# Autodesk Inventor assembly: Assembly2
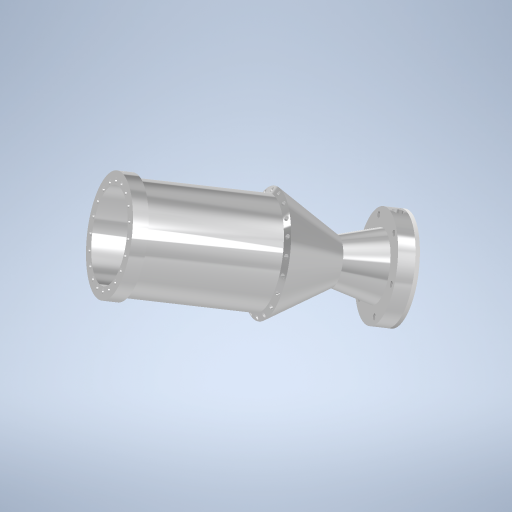
[picture p0: Inventor's stored thumbnail of the model, 512x512]
Saved by Autodesk Inventor 2023 (Build 270158000, 158)
## iProperties
Created: 2022-09-21
Part Number: Assembly2
Document SubType Name: Assembly
Designer: station
Author: station
## Documents named in this file (3)
- C:\Users\station\Documents\Project\Liquid-engine-cooling-system\design files\ethanol engine 6\Assembly2.iam
- C:\Users\station\Documents\Project\Liquid-engine-cooling-system\design files\ethanol engine 6\aluminium engine.ipt
- C:\Users\station\Documents\Project\Liquid-engine-cooling-system\design files\ethanol engine 6\back.ipt
## Components (2 placed, 2 different names)
1. aluminium engine:1 — Mate:1, Mate:2, Mate:3
2. back:1 — Mate:1, Mate:2, Mate:3
## Relationships (3: Mate 3)
- Mate:1: aluminium engine:1 ↔ back:1
- Mate:2: aluminium engine:1 ↔ back:1
- Mate:3: aluminium engine:1 ↔ back:1
